# Autodesk Inventor assembly: ASM_Housing_Bearing_OD
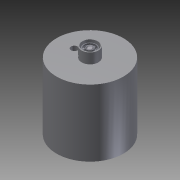
[picture p0: Inventor's stored thumbnail of the model, 180x180]
Saved by Autodesk Inventor 2011 SP2 (Build 150309200, 309)
## iProperties
Created: 2012-02-15
Part Number: ASM_Housing_Bearing_OD
Document SubType Name: Assembly
Designer: sungwook
Author: sungwook
## Documents named in this file (6)
- C:\Users\sungwook\Documents\Inventor\Micron20\Assembly\ASM_Housing_Bearing_OD.iam
- C:\Users\sungwook\Documents\Inventor\Micron20\Parts\Jigs\Bearing_OD_Asm_Base.ipt
- C:\Users\sungwook\Documents\Inventor\Micron20\Parts\Motor Units\MU_Bearing(681h).ipt
- C:\Users\sungwook\Documents\Inventor\Micron20\Parts\Motor Units\MU_Bearing_Retainer.ipt
- C:\Users\sungwook\Documents\Inventor\Micron20\Parts\Motor Units\MU_Motor_Coupling_3.ipt
- C:\Users\sungwook\Documents\Inventor\Micron20\Parts\Motor Units\MU_Motor_Thread.ipt
## Components (5 placed, 5 different names)
1. Bearing_OD_Asm_Base:1 — Mate:3, Mate:8
2. MU_Bearing(681h):1 — Mate:6, Mate:7, Mate:9
3. MU_Bearing_Retainer:1 — Mate:3, Mate:5, Mate:8, Mate:9, Mate:10
4. MU_Motor_Coupling_3:1 — Mate:1, Mate:2, Mate:6, Mate:7, Mate:10
5. MU_Motor_Thread:1 — Mate:1, Mate:2, Mate:5
## Relationships (9: Mate 9)
- Mate:1: MU_Motor_Coupling_3:1 ↔ MU_Motor_Thread:1
- Mate:2: MU_Motor_Coupling_3:1 ↔ MU_Motor_Thread:1
- Mate:3: Bearing_OD_Asm_Base:1 ↔ MU_Bearing_Retainer:1
- Mate:5: MU_Bearing_Retainer:1 ↔ MU_Motor_Thread:1
- Mate:6: MU_Bearing(681h):1 ↔ MU_Motor_Coupling_3:1
- Mate:7: MU_Bearing(681h):1 ↔ MU_Motor_Coupling_3:1
- Mate:8: Bearing_OD_Asm_Base:1 ↔ MU_Bearing_Retainer:1
- Mate:9: MU_Bearing(681h):1 ↔ MU_Bearing_Retainer:1
- Mate:10: MU_Bearing_Retainer:1 ↔ MU_Motor_Coupling_3:1
